# Autodesk Inventor assembly: Battery Module Third Iteration Assembly
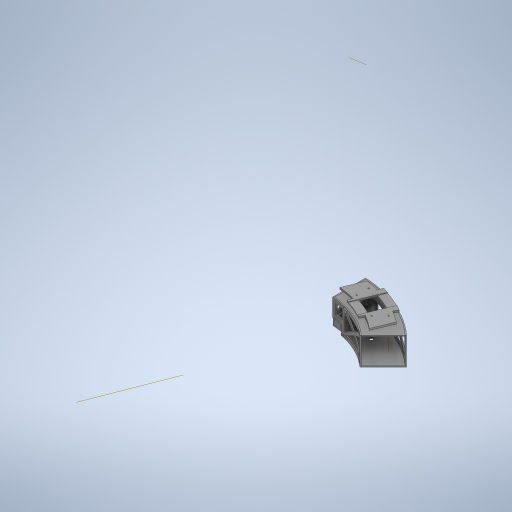
[picture p0: Inventor's stored thumbnail of the model, 512x512]
Saved by Autodesk Inventor 2023 (Build 270158000, 158)
## iProperties
Created: 2023-03-05
Part Number: Battery Module Third Iteration Assembly
Document SubType Name: Assembly
Designer: mihal
Mass: 274.856 g
Surface Area: 1489.36 cm^2
Volume: 219.88 cm^3
Density: 1.25002 g/cm^3
Author: mihal
## Documents named in this file (9)
- C:\Users\mihal\Desktop\4th Year Project\Final Assembly\Battery Module\Battery Module.iam
- C:\Users\mihal\Desktop\4th Year Project\Final Assembly\Battery Module\Battery Module Bottom Plate.ipt
- C:\Users\mihal\Desktop\4th Year Project\Final Assembly\Battery Module\Battery Module Inner Wall.ipt
- C:\Users\mihal\Desktop\4th Year Project\Final Assembly\Battery Module\Battery Module Outer Wall.ipt
- C:\Users\mihal\Desktop\4th Year Project\Final Assembly\Battery Module\Battery Module Top Plate.ipt
- C:\Users\mihal\Desktop\4th Year Project\Final Assembly\Battery Module\Battery Module Back Panel.ipt
- C:\Users\mihal\Desktop\4th Year Project\Final Assembly\Battery Module\Battery Module Top Wing.ipt
- C:\Users\mihal\Desktop\4th Year Project\Final Assembly\Battery Module\Connector Plate.ipt
- C:\Users\mihal\Desktop\4th Year Project\Final Assembly\Battery Module\Female Blade Component.ipt
## Components (15 placed, 8 different names)
1. Battery Module Bottom Plate:1 — Mate:1, Mate:2, Mate:3, Mate:4, Angle:1, Mate:18, Mate:21, Mate:23, Mate:24
2. Battery Module Inner Wall:1 — Mate:1, Mate:2, Mate:11, Mate:16, Mate:19, Mate:20, Mate:26, Mate:31, Mate:32, Mate:33, Mate:34
3. Battery Module Outer Wall:1 — Mate:3, Mate:4, Mate:5, Mate:6, Mate:12, Mate:17, Mate:22, Mate:25, Mate:27, Mate:28, Mate:29, Mate:30
4. Battery Module Top Plate:1 — Mate:5, Mate:6, Mate:8, Mate:9, Mate:10
5. Battery Module Back Panel:1 — Mate:16, Mate:17, Mate:18, Mate:35, Mate:36
6. Battery Module Top Wing:1 — Mate:8, Mate:9, Mate:10, Mate:15
7. Connector Plate:1 — Mate:23, Mate:25
8. Connector Plate:2 — Mate:21, Mate:22
9. Connector Plate:3 — Mate:24, Mate:26
10. Connector Plate:4 — Mate:19, Mate:20
11. Connector Plate:5 — Mate:27, Mate:28
12. Connector Plate:6 — Mate:31, Mate:32
13. Connector Plate:7 — Mate:33, Mate:34
14. Connector Plate:8 — Mate:29, Mate:30
15. Female Blade Component:1 — Mate:35, Mate:36
## Relationships (34: Mate 33, Angle 1)
- Mate:1: Battery Module Bottom Plate:1 ↔ Battery Module Inner Wall:1
- Mate:2: Battery Module Bottom Plate:1 ↔ Battery Module Inner Wall:1
- Mate:3: Battery Module Bottom Plate:1 ↔ Battery Module Outer Wall:1
- Mate:4: Battery Module Bottom Plate:1 ↔ Battery Module Outer Wall:1
- Mate:5: Battery Module Outer Wall:1 ↔ Battery Module Top Plate:1
- Mate:6: Battery Module Outer Wall:1 ↔ Battery Module Top Plate:1
- Mate:8: Battery Module Top Plate:1 ↔ Battery Module Top Wing:1
- Mate:9: Battery Module Top Plate:1 ↔ Battery Module Top Wing:1
- Mate:10: Battery Module Top Plate:1 ↔ Battery Module Top Wing:1
- Mate:11: Battery Module Inner Wall:1
- Mate:12: Battery Module Outer Wall:1
- Mate:15: Battery Module Top Wing:1
- Angle:1 (0 deg): Battery Module Bottom Plate:1
- Mate:16: Battery Module Inner Wall:1 ↔ Battery Module Back Panel:1
- Mate:17: Battery Module Outer Wall:1 ↔ Battery Module Back Panel:1
- Mate:18: Battery Module Bottom Plate:1 ↔ Battery Module Back Panel:1
- Mate:19: Battery Module Inner Wall:1 ↔ Connector Plate:4
- Mate:20: Battery Module Inner Wall:1 ↔ Connector Plate:4
- Mate:21: Battery Module Bottom Plate:1 ↔ Connector Plate:2
- Mate:22: Battery Module Outer Wall:1 ↔ Connector Plate:2
- Mate:23: Battery Module Bottom Plate:1 ↔ Connector Plate:1
- Mate:24: Battery Module Bottom Plate:1 ↔ Connector Plate:3
- Mate:25: Battery Module Outer Wall:1 ↔ Connector Plate:1
- Mate:26: Battery Module Inner Wall:1 ↔ Connector Plate:3
- Mate:27: Battery Module Outer Wall:1 ↔ Connector Plate:5
- Mate:28: Battery Module Outer Wall:1 ↔ Connector Plate:5
- Mate:29: Battery Module Outer Wall:1 ↔ Connector Plate:8
- Mate:30: Battery Module Outer Wall:1 ↔ Connector Plate:8
- Mate:31: Battery Module Inner Wall:1 ↔ Connector Plate:6
- Mate:32: Battery Module Inner Wall:1 ↔ Connector Plate:6
- Mate:33: Battery Module Inner Wall:1 ↔ Connector Plate:7
- Mate:34: Battery Module Inner Wall:1 ↔ Connector Plate:7
- Mate:35: Battery Module Back Panel:1 ↔ Female Blade Component:1
- Mate:36: Battery Module Back Panel:1 ↔ Female Blade Component:1
